# Autodesk Inventor assembly: left pneumatics board
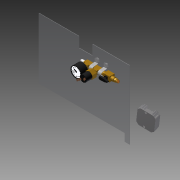
[picture p0: Inventor's stored thumbnail of the model, 180x180]
Saved by Autodesk Inventor 2014 (Build 180170000, 170)
## iProperties
Created: 2014-01-20
Part Number: left pneumatics board
Document SubType Name: Assembly
Designer: Arpan
Author: Arpan
## Documents named in this file (5)
- C:\Users\Andrew Toennies\Documents\GitHub\2014buildCAD\pneumatics board\left pneumatics board.iam
- C:\Users\Andrew Toennies\Documents\GitHub\2014buildCAD\pneumatics board\pneumatics board 1.ipt
- C:\Users\Andrew Toennies\Documents\GitHub\2014buildCAD\pneumatics board\pneumatic thing 1.iam
- C:\Users\Andrew Toennies\Documents\GitHub\2014buildCAD\electrical\CS_Converter_CLL25-24S05.ipt
- C:\Users\Andrew Toennies\Documents\GitHub\2014buildCAD\electrical\CS_WirelessBridge_DAP1522.ipt
## Components (4 placed, 4 different names)
1. pneumatics board 1:1 — Mate:1, Mate:4, Flush:3, Flush:4, Flush:5, Flush:6, Mate:5, Mate:7, Mate:8
2. pneumatic thing 1:1 [sub-assembly] — Mate:1, Flush:5, Flush:6
3. CS_Converter_CLL25-24S05:1 — Mate:5, Mate:7, Mate:8
4. CS_WirelessBridge_DAP1522:1 — Mate:4, Flush:3, Flush:4
## Relationships (9: Mate 5, Flush 4)
- Mate:1: pneumatics board 1:1 ↔ pneumatic thing 1:1
- Mate:4: pneumatics board 1:1 ↔ CS_WirelessBridge_DAP1522:1
- Flush:3 (12.7 mm): pneumatics board 1:1 ↔ CS_WirelessBridge_DAP1522:1
- Flush:4 (12.7 mm): pneumatics board 1:1 ↔ CS_WirelessBridge_DAP1522:1
- Flush:5 (50.8 mm): pneumatics board 1:1 ↔ pneumatic thing 1:1
- Flush:6 (25.4 mm): pneumatics board 1:1 ↔ pneumatic thing 1:1
- Mate:5: pneumatics board 1:1 ↔ CS_Converter_CLL25-24S05:1
- Mate:7 (203.2 mm): pneumatics board 1:1 ↔ CS_Converter_CLL25-24S05:1
- Mate:8: pneumatics board 1:1 ↔ CS_Converter_CLL25-24S05:1
